# Autodesk Inventor assembly: Satellite Droit
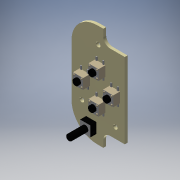
[picture p0: Inventor's stored thumbnail of the model, 180x180]
Saved by Autodesk Inventor 2016 SP1 (Build 200210100, 210)
## iProperties
Created: 2018-06-08
Part Number: Satellite Droit
Material: Générique
Document SubType Name: Assembly
Designer: dimercur
Author: dimercur
## Documents named in this file (4)
- D:\Users\dimercur\Documents\git\arm-ada-ng\hardware\Box\Satellite Droit.iam
- D:\Users\dimercur\Documents\git\arm-ada-ng\hardware\Box\PCB Droit.ipt
- D:\Users\dimercur\Documents\git\arm-ada-ng\hardware\Box\Touch Button.ipt
- D:\Users\dimercur\Documents\git\arm-ada-ng\hardware\Box\Touch Button High.ipt
## Components (6 placed, 3 different names)
1. PCB Droit:1 — Placage:1, Placage:2, Placage:3, Placage:4, Placage:5, Placage:6, Placage:7, Placage:8, Placage:9, Placage:10, Placage:11, Placage:12, Placage:13, Placage:14, Placage:15
2. Touch Button:1 — Placage:1, Placage:8, Placage:11
3. Touch Button:2 — Placage:2, Placage:5, Placage:6
4. Touch Button:3 — Placage:3, Placage:7, Placage:10
5. Touch Button:4 — Placage:4, Placage:9, Placage:12
6. Touch Button High:1 — Placage:13, Placage:14, Placage:15
## Relationships (15: Mate 15)
- Placage:1 [Mate]: PCB Droit:1 ↔ Touch Button:1
- Placage:2 [Mate]: PCB Droit:1 ↔ Touch Button:2
- Placage:3 [Mate]: PCB Droit:1 ↔ Touch Button:3
- Placage:4 [Mate]: PCB Droit:1 ↔ Touch Button:4
- Placage:5 [Mate] (10.25 mm): PCB Droit:1 ↔ Touch Button:2
- Placage:6 [Mate] (11.25 mm): PCB Droit:1 ↔ Touch Button:2
- Placage:7 [Mate] (2.75 mm): PCB Droit:1 ↔ Touch Button:3
- Placage:8 [Mate] (20.25 mm): PCB Droit:1 ↔ Touch Button:1
- Placage:9 [Mate] (-11.25 mm): PCB Droit:1 ↔ Touch Button:4
- Placage:10 [Mate] (19.25 mm): PCB Droit:1 ↔ Touch Button:3
- Placage:11 [Mate] (19.25 mm): PCB Droit:1 ↔ Touch Button:1
- Placage:12 [Mate] (28.25 mm): PCB Droit:1 ↔ Touch Button:4
- Placage:13 [Mate]: PCB Droit:1 ↔ Touch Button High:1
- Placage:14 [Mate] (5 mm): PCB Droit:1 ↔ Touch Button High:1
- Placage:15 [Mate] (4 mm): PCB Droit:1 ↔ Touch Button High:1
